# Autodesk Inventor assembly: V4.0-trebuchet-printable
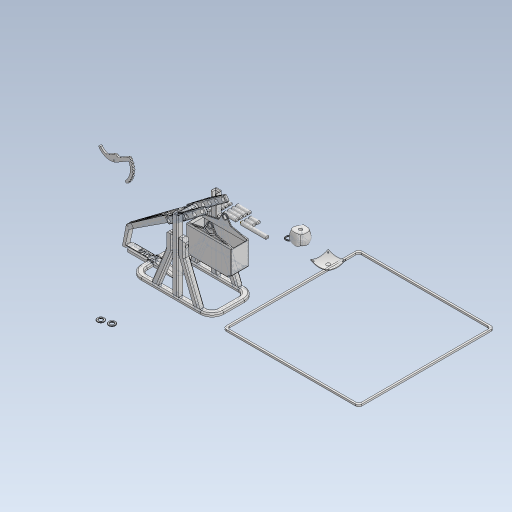
[picture p0: Inventor's stored thumbnail of the model, 512x512]
Saved by Autodesk Inventor 2023 (Build 270158030, 158C)
## iProperties
Created: 2024-12-20
Part Number: V4.0-trebuchet-printable
Document SubType Name: Assembly
Designer: Imogen Heard
Author: Imogen Heard
## Documents named in this file (23)
- C:\Users\dheard\Documents\0004-inventor\3D-CAD-main\trebuchet\V4.0-trebuchet-printable.iam
- C:\Users\dheard\Documents\0004-inventor\3D-CAD-main\trebuchet\pins.ipt
- C:\Users\dheard\Documents\0004-inventor\3D-CAD-main\trebuchet\bolder.ipt
- C:\Users\dheard\Documents\0004-inventor\3D-CAD-main\trebuchet\sling.ipt
- C:\Users\dheard\Documents\0004-inventor\3D-CAD-main\unicorn-horn\washers.ipt
- C:\Users\dheard\Documents\0004-inventor\3D-CAD-main\trebuchet\throw-ring.ipt
- C:\Users\dheard\Documents\0004-inventor\3D-CAD-main\trebuchet\border.ipt
- C:\Users\dheard\Documents\0004-inventor\3D-CAD-main\trebuchet\baseplate.ipt
- C:\Users\dheard\Documents\0004-inventor\3D-CAD-main\trebuchet\V4-upright-A.ipt
- C:\Users\dheard\Documents\0004-inventor\3D-CAD-main\trebuchet\V4-a-frame-A.ipt
- C:\Users\dheard\Documents\0004-inventor\3D-CAD-main\trebuchet\V4-pivot-A.ipt
- C:\Users\dheard\Documents\0004-inventor\3D-CAD-main\trebuchet\V4-throw-arm.ipt
- C:\Users\dheard\Documents\0004-inventor\3D-CAD-main\trebuchet\V4-ratchet.ipt
- C:\Users\dheard\Documents\0004-inventor\3D-CAD-main\trebuchet\V4-counterweight.ipt
- C:\Users\dheard\Documents\0004-inventor\3D-CAD-main\trebuchet\V4-pivot-B.ipt
- C:\Users\dheard\Documents\0004-inventor\3D-CAD-main\trebuchet\V4-upright-B.ipt
- C:\Users\dheard\Documents\0004-inventor\3D-CAD-main\trebuchet\V4-a-frame-B.ipt
- C:\Users\dheard\Documents\0004-inventor\3D-CAD-main\trebuchet\V4-a-frame-C.ipt
- C:\Users\dheard\Documents\0004-inventor\3D-CAD-main\trebuchet\V4-a-frame-D.ipt
- C:\Users\dheard\Documents\0004-inventor\3D-CAD-main\trebuchet\V4-spacer-A.ipt
- C:\Users\dheard\Documents\0004-inventor\3D-CAD-main\trebuchet\V4-spacer-B.ipt
- C:\Users\dheard\Documents\0004-inventor\3D-CAD-main\trebuchet\v4-latch.ipt
- C:\Users\dheard\Documents\0004-inventor\3D-CAD-main\trebuchet\V4-pegs.ipt
## Components (23 placed, 22 different names)
1. pins:1 — Flush:7, Flush:25, Flush:26, Flush:27, Flush:28, Flush:29, Flush:30, Flush:31, Flush:32, Flush:33, Flush:34, Flush:35, Flush:36, Flush:37, Flush:38, Flush:39
2. bolder:1 — Flush:41
3. sling:1 — Flush:40
4. washers:1 — Flush:19
5. washers:2 — Flush:21
6. throw-ring:1 — Flush:18
7. border:1 — Flush:7, Flush:18, Flush:19, Flush:21, Flush:25, Flush:26, Flush:27, Flush:28, Flush:29, Flush:30, Flush:31, Flush:32, Flush:33, Flush:34, Flush:35, Flush:36, Flush:37, Flush:38, Flush:39, Flush:40, Flush:41, Flush:42
8. V4-baseplate:1 — Flush:42, Flush:43
9. V4-upright-A:1 — Rotational:1
10. V4-a-frame-A:1
11. V4-pivot-A:1 — Rotational:1, Insert:1, Insert:2
12. V4-throw-arm:1 — Insert:3, Insert:4, Insert:6, Insert:7
13. V4-ratchet:1
14. V4-counterweight:1
15. V4-pivot-B:1 — Insert:5, Insert:8
16. V4-upright-B:1
17. V4-a-frame-B:1
18. V4-a-frame-C:1
19. V4-a-frame-D:1
20. V4-spacer-A:1 — Insert:1, Insert:2, Insert:3, Insert:4
21. V4-spacer-B:1 — Insert:5, Insert:6, Insert:7, Insert:8
22. v4-latch:1 — Flush:43, Flush:44
23. V4-pegs:1 — Flush:44
## Relationships (33: Flush 24, Insert 8, RevoluteJoint 1)
- Flush:7: pins:1 ↔ border:1
- Flush:18: throw-ring:1 ↔ border:1
- Flush:19: washers:1 ↔ border:1
- Flush:21: washers:2 ↔ border:1
- Flush:25: pins:1 ↔ border:1
- Flush:26: pins:1 ↔ border:1
- Flush:27: pins:1 ↔ border:1
- Flush:28: pins:1 ↔ border:1
- Flush:29: pins:1 ↔ border:1
- Flush:30: pins:1 ↔ border:1
- Flush:31: pins:1 ↔ border:1
- Flush:32: pins:1 ↔ border:1
- Flush:33: pins:1 ↔ border:1
- Flush:34: pins:1 ↔ border:1
- Flush:35: pins:1 ↔ border:1
- Flush:36: pins:1 ↔ border:1
- Flush:37: pins:1 ↔ border:1
- Flush:38: pins:1 ↔ border:1
- Flush:39: pins:1 ↔ border:1
- Flush:40: sling:1 ↔ border:1
- Flush:41: bolder:1 ↔ border:1
- Flush:42: border:1 ↔ V4-baseplate:1
- Rotational:1 [RevoluteJoint] (-5.4 mm): V4-upright-A:1 ↔ V4-pivot-A:1
- Insert:1: V4-pivot-A:1 ↔ V4-spacer-A:1
- Insert:2: V4-pivot-A:1 ↔ V4-spacer-A:1
- Insert:3: V4-throw-arm:1 ↔ V4-spacer-A:1
- Insert:4: V4-throw-arm:1 ↔ V4-spacer-A:1
- Insert:5: V4-pivot-B:1 ↔ V4-spacer-B:1
- Insert:6: V4-throw-arm:1 ↔ V4-spacer-B:1
- Insert:7: V4-throw-arm:1 ↔ V4-spacer-B:1
- Insert:8: V4-pivot-B:1 ↔ V4-spacer-B:1
- Flush:43: V4-baseplate:1 ↔ v4-latch:1
- Flush:44: v4-latch:1 ↔ V4-pegs:1
